# Autodesk Inventor assembly: wheel_with_mounts
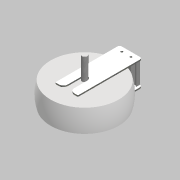
[picture p0: Inventor's stored thumbnail of the model, 180x180]
Saved by Autodesk Inventor 2021.2 (Build 252289000, 289)
## iProperties
Created: 2021-05-27
Part Number: wheel_with_mounts
Document SubType Name: Assembly
Designer: gisen
Author: gisen
## Documents named in this file (4)
- C:\Users\gisen\workspace\beetle_inventor_model\suspension\wheel_with_mounts.iam
- C:\Users\gisen\workspace\beetle_inventor_model\suspension\6inch_wheel.ipt
- C:\Users\gisen\workspace\beetle_inventor_model\suspension\wheel_mount.ipt
- C:\Users\gisen\workspace\beetle_inventor_model\suspension\AFS-2040-4-50.ipt
## Components (4 placed, 3 different names)
1. 6inch_wheel:1 — メイト:1, メイト:2, メイト:3, フラッシュ:3, フラッシュ:2, フラッシュ:10, メイト:12
2. wheel_mount — メイト:3, フラッシュ:3, メイト:4, フラッシュ:11, フラッシュ:10, フラッシュ:12, メイト:12
3. wheel_mount:2 — メイト:9, メイト:10, メイト:11
4. AFS-2040-4-50:1 — メイト:4, フラッシュ:11, フラッシュ:2, メイト:9, メイト:10, メイト:11
## Relationships (13: Mate 8, Flush 5)
- メイト:1 [Mate]: 6inch_wheel:1
- メイト:2 [Mate]: 6inch_wheel:1
- メイト:3 [Mate]: 6inch_wheel:1 ↔ wheel_mount
- フラッシュ:3 [Flush]: 6inch_wheel:1 ↔ wheel_mount
- メイト:4 [Mate]: wheel_mount ↔ AFS-2040-4-50:1
- フラッシュ:11 [Flush]: wheel_mount ↔ AFS-2040-4-50:1
- フラッシュ:2 [Flush]: 6inch_wheel:1 ↔ AFS-2040-4-50:1
- フラッシュ:10 [Flush]: 6inch_wheel:1 ↔ wheel_mount
- メイト:9 [Mate]: wheel_mount:2 ↔ AFS-2040-4-50:1
- メイト:10 [Mate]: wheel_mount:2 ↔ AFS-2040-4-50:1
- メイト:11 [Mate]: wheel_mount:2 ↔ AFS-2040-4-50:1
- フラッシュ:12 [Flush]: wheel_mount
- メイト:12 [Mate]: 6inch_wheel:1 ↔ wheel_mount
